# Autodesk Inventor assembly: 1892mm
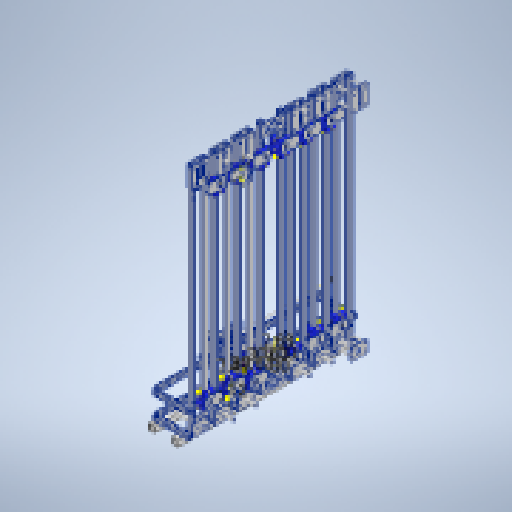
[picture p0: Inventor's stored thumbnail of the model, 512x512]
Saved by Autodesk Inventor 2025 (Build 290162000, 162)
## iProperties
Created: 2025-02-24
Part Number: 1892mm
Document SubType Name: Assembly
Designer: Zhopa
Mass: 1645.37 g
Surface Area: 12511.3 cm^2
Volume: 1061.14 cm^3
Author: Zhopa
## Documents named in this file (24)
- C:\Users\onion\OneDrive - Kyushu University\共有用\工房共有ワンドライブ2024~2025用\ハード\NHK2025\onitsuka\p_a_g\Workspace\Vova\elevator 3\1892mm.iam
- C:\Users\onion\OneDrive - Kyushu University\共有用\工房共有ワンドライブ2024~2025用\ハード\NHK2025\Vova\elevator 3\beams\10x10x600.ipt
- C:\Users\onion\OneDrive - Kyushu University\共有用\工房共有ワンドライブ2024~2025用\ハード\NHK2025\Vova\elevator 3\3D printed\filler_side_fix.ipt
- C:\Users\onion\OneDrive - Kyushu University\共有用\工房共有ワンドライブ2024~2025用\ハード\NHK2025\Vova\elevator 3\cnc\2mm_double_for_pulley.ipt
- C:\Users\onion\OneDrive - Kyushu University\共有用\工房共有ワンドライブ2024~2025用\ハード\NHK2025\Vova\elevator 3\beams\Ф8x40.ipt
- C:\Users\onion\OneDrive - Kyushu University\共有用\工房共有ワンドライブ2024~2025用\ハード\NHK2025\Vova\elevator 3\cnc\2mm_double_for_pulley_v1.ipt
- C:\Users\onion\OneDrive - Kyushu University\共有用\工房共有ワンドライブ2024~2025用\ハード\NHK2025\Vova\elevator 3\cnc\belt_holder_1.ipt
- C:\Users\onion\OneDrive - Kyushu University\共有用\工房共有ワンドライブ2024~2025用\ハード\NHK2025\Vova\elevator 3\cnc\belt_holder_2.ipt
- C:\Users\onion\OneDrive - Kyushu University\共有用\工房共有ワンドライブ2024~2025用\ハード\NHK2025\Vova\elevator 3\cnc\2mm_double_for_pulley_v1_center.ipt
- C:\Users\onion\OneDrive - Kyushu University\共有用\工房共有ワンドライブ2024~2025用\ハード\NHK2025\Vova\elevator 3\bearings\DDLF-1280ZZ.ipt
- C:\Users\onion\OneDrive - Kyushu University\共有用\工房共有ワンドライブ2024~2025用\ハード\NHK2025\Vova\elevator 3\subassemblies\carriage+holder_short.iam
- C:\Users\onion\OneDrive - Kyushu University\共有用\工房共有ワンドライブ2024~2025用\ハード\NHK2025\Vova\elevator 3\beams\10x10x600 - Copy.ipt
- C:\Users\onion\OneDrive - Kyushu University\共有用\工房共有ワンドライブ2024~2025用\ハード\NHK2025\Vova\elevator 3\beams\10x10x60.ipt
- C:\Users\onion\OneDrive - Kyushu University\共有用\工房共有ワンドライブ2024~2025用\ハード\NHK2025\Vova\elevator 3\beams\10x10x431.ipt
- C:\Users\onion\OneDrive - Kyushu University\共有用\工房共有ワンドライブ2024~2025用\ハード\NHK2025\Vova\elevator 3\cnc\motor.ipt
- C:\Users\onion\OneDrive - Kyushu University\共有用\工房共有ワンドライブ2024~2025用\ハード\NHK2025\Vova\elevator 3\motor\M3508.ipt
- C:\Users\onion\OneDrive - Kyushu University\共有用\工房共有ワンドライブ2024~2025用\ハード\NHK2025\Vova\elevator 3\motor\C620.ipt
- C:\Users\onion\OneDrive - Kyushu University\共有用\工房共有ワンドライブ2024~2025用\ハード\NHK2025\Vova\elevator 3\cnc\motor - Copy (2).ipt
- C:\Users\onion\OneDrive - Kyushu University\共有用\工房共有ワンドライブ2024~2025用\ハード\NHK2025\Vova\elevator 3\subassemblies\full short almost works - Copy\Design Accelerator\Spur Gears2.iam
- C:\Users\onion\OneDrive - Kyushu University\共有用\工房共有ワンドライブ2024~2025用\ハード\NHK2025\Vova\elevator 3\beams\Ф8x77.ipt
- C:\Users\onion\OneDrive - Kyushu University\共有用\工房共有ワンドライブ2024~2025用\ハード\NHK2025\Vova\elevator 3\subassemblies\tension.iam
- C:\Users\onion\OneDrive - Kyushu University\共有用\工房共有ワンドライブ2024~2025用\ハード\NHK2025\Vova\elevator 3\cnc\motor - Copy (2) - Copy.ipt
- C:\Users\onion\OneDrive - Kyushu University\共有用\工房共有ワンドライブ2024~2025用\ハード\NHK2025\Vova\elevator 3\3D printed\sapcer34mm.ipt
- C:\Users\onion\OneDrive - Kyushu University\共有用\工房共有ワンドライブ2024~2025用\ハード\NHK2025\Vova\elevator 3\beams\15x15x455.ipt
## Components (101 placed, 23 different names)
1. 10x10x600:9 — 挿入:5, 正接:7, 正接:8, 正接:9, 正接:10, 正接:11, 正接:12, スライダ:1, 挿入:229, 挿入:230, 挿入:231, 挿入:232, 挿入:233, 挿入:234, 挿入:235, 挿入:236
2. filler_side_fix:1 — 挿入:213, 挿入:214
3. filler_side_fix:2 — 挿入:5, 挿入:215, 挿入:216
4. filler_side_fix:3 — 挿入:170, 挿入:171, 挿入:217, 挿入:218
5. filler_side_fix:4 — 挿入:219, 挿入:220
6. 10x10x600:3 — 挿入:24, 挿入:25, 挿入:26, 挿入:27, 挿入:28, 挿入:48, 挿入:49, 挿入:55, 挿入:56, 挿入:58, スライダ:1, 正接:40, 正接:41, 正接:42, 正接:43
7. carriage+holder_short:1 [sub-assembly] — 挿入:24, 挿入:25, 挿入:26, 挿入:27, 正接:7, 正接:8, 正接:9, 正接:10, 正接:11, 正接:12, 挿入:29, 挿入:30, 挿入:31, 挿入:32, 挿入:71, 挿入:72
8. filler_side_fix:5 — 挿入:28, 挿入:29, 挿入:30
9. filler_side_fix:6 — 挿入:31, 挿入:32
10. 2mm_double_for_pulley:1 — 挿入:48, 挿入:168, 挿入:169
11. 2mm_double_for_pulley:2 — 挿入:49, 挿入:51, 挿入:176
12. Ф8x40:1 — 挿入:51
13. 2mm_double_for_pulley_v1:1 — 挿入:55, 挿入:56, 挿入:135, 挿入:172, 挿入:174
14. 2mm_double_for_pulley_v1:2 — 挿入:58, 挿入:60, 挿入:134, 挿入:173, 挿入:175
15. Ф8x40:2 — 挿入:60
16. Ф8x40:3 — 正接:62, 正接:76
17. belt_holder_1:1 — 挿入:71, 挿入:72, 挿入:73, 挿入:74
18. belt_holder_2:1 — 挿入:73, 挿入:74
19. belt_holder_1:2
20. belt_holder_2:2
21. 2mm_double_for_pulley_v1_center:1 — 挿入:182, 挿入:184, 挿入:190, 挿入:192
22. 10x10x600:6 — スライダ:4, 挿入:205, 挿入:206, 挿入:207, 挿入:208, 正接:52, 正接:53, 正接:54, 正接:55
23. 2mm_double_for_pulley:5 — 挿入:198, 挿入:200
24. 2mm_double_for_pulley:6 — 挿入:197, 挿入:199
25. Ф8x40:6
26. 2mm_double_for_pulley_v1:5 — 挿入:138, 挿入:193, 挿入:196
27. 2mm_double_for_pulley_v1:6 — 挿入:140, 挿入:194, 挿入:195
28. Ф8x40:7
29. 10x10x600:8 — スライダ:4, 正接:32, 正接:33, 正接:34, 正接:35, 挿入:225, 挿入:226, 挿入:227, 挿入:228, 挿入:245, 挿入:246, 挿入:247, 挿入:248, 挿入:253, 挿入:254, 挿入:258
30. Ф8x40:9 — 正接:61, 正接:63, 正接:64
31. DDLF-1280ZZ:3 — 挿入:134
32. DDLF-1280ZZ:4 — 挿入:135
33. DDLF-1280ZZ:7 — 挿入:138
34. DDLF-1280ZZ:8 — 挿入:140
35. 2mm_double_for_pulley_v1_center:2 — 挿入:181, 挿入:183, 挿入:189, 挿入:191
36. Ф8x40:13 — 正接:61, 挿入:259
37. 10x10x600 - Copy:1 — 挿入:168, 挿入:169, 挿入:170, 挿入:171, 挿入:172, 挿入:173, 挿入:174, 挿入:175, 挿入:176, 正接:28, 正接:29, 正接:30, 正接:31, 挿入:218, スライダ:5
38. 10x10x600 - Copy:2 — 挿入:181, 挿入:182, 挿入:183, 挿入:184, 挿入:201, 挿入:202, 挿入:203, 挿入:204, 正接:44, 正接:45, 正接:46, 正接:47, スライダ:5
39. 10x10x600 - Copy:3 — 挿入:189, 挿入:190, 挿入:191, 挿入:192, 挿入:209, 挿入:210, 挿入:211, 挿入:212, 正接:48, 正接:49, 正接:50, 正接:51
40. 10x10x600 - Copy:4 — 挿入:193, 挿入:194, 挿入:195, 挿入:196, 挿入:197, 挿入:198, 挿入:199, 挿入:200, 正接:36, 正接:37, 正接:38, 正接:39, 挿入:221, 挿入:222, 挿入:223, 挿入:224
41. carriage+holder_short:2 [sub-assembly] — 挿入:201, 挿入:202, 挿入:203, 挿入:204, 正接:28, 正接:29, 正接:30, 正接:31
42. carriage+holder_short:3 [sub-assembly] — 挿入:205, 挿入:206, 挿入:207, 挿入:208, 正接:32, 正接:33, 正接:34, 正接:35
43. carriage+holder_short:4 [sub-assembly] — 挿入:209, 挿入:210, 挿入:211, 挿入:212, 正接:36, 正接:37, 正接:38, 正接:39
44. carriage+holder_short:5 [sub-assembly] — 挿入:213, 挿入:214, 挿入:215, 挿入:216, 正接:40, 正接:41, 正接:42, 正接:43
45. carriage+holder_short:6 [sub-assembly] — 挿入:217, 挿入:219, 挿入:220, 正接:44, 正接:45, 正接:46, 正接:47
46. carriage+holder_short:7 [sub-assembly] — 挿入:221, 挿入:222, 挿入:223, 挿入:224, 正接:48, 正接:49, 正接:50, 正接:51
47. carriage+holder_short:8 [sub-assembly] — 挿入:225, 挿入:226, 挿入:227, 挿入:228, 正接:52, 正接:53, 正接:54, 正接:55
48. 2mm_double_for_pulley:7 — 挿入:229, 挿入:230, 正接:62, 挿入:237, 挿入:238
49. 2mm_double_for_pulley:8 — 挿入:231, 挿入:232, 挿入:239, 挿入:240
50. 2mm_double_for_pulley_v1:7 — 挿入:233, 挿入:234, 挿入:243, 挿入:244
51. 2mm_double_for_pulley_v1:8 — 挿入:235, 挿入:236, 挿入:241, 挿入:242, 挿入:340
52. 10x10x600:10 — 挿入:237, 挿入:238, 挿入:239, 挿入:240, 挿入:241, 挿入:242, 挿入:243, 挿入:244, 挿入:280, 挿入:281, 挿入:282, 挿入:283, スライダ:6
53. 2mm_double_for_pulley:9 — 挿入:245, 挿入:246, 正接:64, 挿入:249, 挿入:250
54. 2mm_double_for_pulley:10 — 挿入:247, 挿入:248, 正接:63, 挿入:251, 挿入:252
55. 10x10x600:11 — 挿入:249, 挿入:250, 挿入:251, 挿入:252, 挿入:255, 挿入:256, 挿入:257, 挿入:307, 挿入:308, 挿入:309, 挿入:310, スライダ:7
56. 2mm_double_for_pulley_v1:9 — 挿入:253, 挿入:254, 挿入:255, 挿入:256
57. 2mm_double_for_pulley_v1:10 — 挿入:257, 挿入:258, 挿入:259
58. 10x10x600:12 — 挿入:284, 挿入:285, 挿入:286, 挿入:287, スライダ:6, 挿入:336, 挿入:337
59. carriage+holder_short:9 [sub-assembly] — 挿入:280, 挿入:281, 挿入:282, 挿入:283
60. 2mm_double_for_pulley_v1:11
61. 2mm_double_for_pulley_v1:12 — 挿入:334
62. 10x10x600:13 — 挿入:314, 挿入:335, 挿入:338, メイト:3, 角度:1
63. carriage+holder_short:11 [sub-assembly] — 挿入:284, 挿入:285, 挿入:286, 挿入:287
64. 10x10x600:14 — 挿入:292, 挿入:293, 挿入:300, 挿入:301, スライダ:7, 挿入:345, 挿入:346, 挿入:348, 挿入:350
65. Ф8x77:1 — 挿入:306
66. carriage+holder_short:12 [sub-assembly] — 挿入:307, 挿入:308, 挿入:309, 挿入:310
67. carriage+holder_short:13 [sub-assembly]
68. 2mm_double_for_pulley:13 — 挿入:292, 挿入:293, 挿入:296, 挿入:297
69. 2mm_double_for_pulley:14
70. 10x10x600:15 — 挿入:296, 挿入:297, 挿入:302, 挿入:303, 挿入:311, 挿入:312, 挿入:343, 挿入:344, 挿入:347, 挿入:349
71. 2mm_double_for_pulley_v1:13 — 挿入:300, 挿入:301, 挿入:302, 挿入:303
72. 2mm_double_for_pulley_v1:14 — 挿入:306
73. 10x10x60:3 — 挿入:311, 挿入:320, 挿入:352, 挿入:358
74. 10x10x60:4 — 挿入:312, 挿入:353
75. 10x10x60:6 — 挿入:314, 挿入:354, 角度:1
76. motor:1 — 挿入:321, 挿入:322, 挿入:328, 挿入:330, メイト:4, 挿入:355, 挿入:356
77. 10x10x431:2 — 挿入:320, 挿入:342
78. M3508:1 — 挿入:321, 挿入:322, メイト:1
79. C620:1
80. DDLF-1280ZZ:13 — 挿入:328
81. motor - Copy (2):1 — 挿入:330, 挿入:331, 挿入:355
82. DDLF-1280ZZ:14 — 挿入:331
83. Spur Gears:1 [sub-assembly] — メイト:1
84. Ф8x77:2
85. Ф8x77:3 — 挿入:334
86. tension:1 [sub-assembly] — 挿入:335, 挿入:336
87. tension:2 [sub-assembly] — 挿入:337, 挿入:338
88. motor - Copy (2) - Copy:1 — 挿入:356
89. Ф8x40:14 — 挿入:340, 正接:76
90. 10x10x60:7 — 挿入:342, メイト:3, 挿入:351, 挿入:357
91. sapcer34mm:1 — 挿入:343
92. sapcer34mm:2 — 挿入:344
93. sapcer34mm:3 — 挿入:345
94. sapcer34mm:4 — 挿入:346
95. sapcer34mm:5 — 挿入:350
96. sapcer34mm:6 — 挿入:349
97. sapcer34mm:7 — 挿入:348
98. sapcer34mm:8 — 挿入:347
99. 15x15x455:1 — 挿入:351, 挿入:352
100. 10x10x431:3 — 挿入:353, 挿入:354, メイト:4
101. 15x15x455:2 — 挿入:357, 挿入:358
## Relationships (248: Insert 189, Tangent 49, TranslationJoint 5, Mate 4, Angle 1)
- 挿入:5 [Insert]: 10x10x600:9 ↔ filler_side_fix:2
- 挿入:24 [Insert] (8 mm): 10x10x600:3 ↔ carriage+holder_short:1
- 挿入:25 [Insert] (8 mm): 10x10x600:3 ↔ carriage+holder_short:1
- 挿入:26 [Insert] (8 mm): 10x10x600:3 ↔ carriage+holder_short:1
- 挿入:27 [Insert] (8 mm): 10x10x600:3 ↔ carriage+holder_short:1
- 正接:7 [Tangent]: 10x10x600:9 ↔ carriage+holder_short:1
- 正接:8 [Tangent]: 10x10x600:9 ↔ carriage+holder_short:1
- 正接:9 [Tangent]: 10x10x600:9 ↔ carriage+holder_short:1
- 正接:10 [Tangent]: 10x10x600:9 ↔ carriage+holder_short:1
- 正接:11 [Tangent]: 10x10x600:9 ↔ carriage+holder_short:1
- 正接:12 [Tangent]: 10x10x600:9 ↔ carriage+holder_short:1
- 挿入:28 [Insert]: 10x10x600:3 ↔ filler_side_fix:5
- 挿入:29 [Insert]: carriage+holder_short:1 ↔ filler_side_fix:5
- 挿入:30 [Insert]: carriage+holder_short:1 ↔ filler_side_fix:5
- 挿入:31 [Insert]: carriage+holder_short:1 ↔ filler_side_fix:6
- 挿入:32 [Insert]: carriage+holder_short:1 ↔ filler_side_fix:6
- 挿入:48 [Insert]: 10x10x600:3 ↔ 2mm_double_for_pulley:1
- 挿入:49 [Insert]: 10x10x600:3 ↔ 2mm_double_for_pulley:2
- 挿入:51 [Insert] (-2 mm): 2mm_double_for_pulley:2 ↔ Ф8x40:1
- 挿入:55 [Insert]: 10x10x600:3 ↔ 2mm_double_for_pulley_v1:1
- 挿入:56 [Insert]: 10x10x600:3 ↔ 2mm_double_for_pulley_v1:1
- 挿入:58 [Insert]: 10x10x600:3 ↔ 2mm_double_for_pulley_v1:2
- 挿入:60 [Insert]: 2mm_double_for_pulley_v1:2 ↔ Ф8x40:2
- 挿入:71 [Insert]: carriage+holder_short:1 ↔ belt_holder_1:1
- 挿入:72 [Insert]: carriage+holder_short:1 ↔ belt_holder_1:1
- 挿入:73 [Insert] (2 mm): belt_holder_1:1 ↔ belt_holder_2:1
- 挿入:74 [Insert] (2 mm): belt_holder_1:1 ↔ belt_holder_2:1
- [Insert] (2 mm): belt_holder_1:2 ↔ belt_holder_2:2
- [Insert] (2 mm): belt_holder_1:2 ↔ belt_holder_2:2
- [Insert]: 10x10x600:6 ↔ 2mm_double_for_pulley:5
- [Insert]: 10x10x600:6 ↔ 2mm_double_for_pulley:6
- [Insert] (-2 mm): 2mm_double_for_pulley:6 ↔ Ф8x40:6
- [Insert]: 10x10x600:6 ↔ 2mm_double_for_pulley_v1:5
- [Insert]: 10x10x600:6 ↔ 2mm_double_for_pulley_v1:6
- [Insert]: 2mm_double_for_pulley_v1:6 ↔ Ф8x40:7
- 挿入:134 [Insert]: 2mm_double_for_pulley_v1:2 ↔ DDLF-1280ZZ:3
- 挿入:135 [Insert]: 2mm_double_for_pulley_v1:1 ↔ DDLF-1280ZZ:4
- 挿入:138 [Insert]: 2mm_double_for_pulley_v1:5 ↔ DDLF-1280ZZ:7
- 挿入:140 [Insert]: 2mm_double_for_pulley_v1:6 ↔ DDLF-1280ZZ:8
- 挿入:168 [Insert]: 2mm_double_for_pulley:1 ↔ 10x10x600 - Copy:1
- 挿入:169 [Insert]: 2mm_double_for_pulley:1 ↔ 10x10x600 - Copy:1
- 挿入:170 [Insert]: filler_side_fix:3 ↔ 10x10x600 - Copy:1
- 挿入:171 [Insert]: filler_side_fix:3 ↔ 10x10x600 - Copy:1
- 挿入:172 [Insert]: 2mm_double_for_pulley_v1:1 ↔ 10x10x600 - Copy:1
- 挿入:173 [Insert]: 2mm_double_for_pulley_v1:2 ↔ 10x10x600 - Copy:1
- 挿入:174 [Insert]: 2mm_double_for_pulley_v1:1 ↔ 10x10x600 - Copy:1
- 挿入:175 [Insert]: 2mm_double_for_pulley_v1:2 ↔ 10x10x600 - Copy:1
- 挿入:176 [Insert]: 2mm_double_for_pulley:2 ↔ 10x10x600 - Copy:1
- 挿入:181 [Insert]: 2mm_double_for_pulley_v1_center:2 ↔ 10x10x600 - Copy:2
- 挿入:182 [Insert]: 2mm_double_for_pulley_v1_center:1 ↔ 10x10x600 - Copy:2
- 挿入:183 [Insert]: 2mm_double_for_pulley_v1_center:2 ↔ 10x10x600 - Copy:2
- 挿入:184 [Insert]: 2mm_double_for_pulley_v1_center:1 ↔ 10x10x600 - Copy:2
- 挿入:189 [Insert]: 2mm_double_for_pulley_v1_center:2 ↔ 10x10x600 - Copy:3
- 挿入:190 [Insert]: 2mm_double_for_pulley_v1_center:1 ↔ 10x10x600 - Copy:3
- 挿入:191 [Insert]: 2mm_double_for_pulley_v1_center:2 ↔ 10x10x600 - Copy:3
- 挿入:192 [Insert]: 2mm_double_for_pulley_v1_center:1 ↔ 10x10x600 - Copy:3
- 挿入:193 [Insert]: 2mm_double_for_pulley_v1:5 ↔ 10x10x600 - Copy:4
- 挿入:194 [Insert]: 2mm_double_for_pulley_v1:6 ↔ 10x10x600 - Copy:4
- 挿入:195 [Insert]: 2mm_double_for_pulley_v1:6 ↔ 10x10x600 - Copy:4
- 挿入:196 [Insert]: 2mm_double_for_pulley_v1:5 ↔ 10x10x600 - Copy:4
- 挿入:197 [Insert]: 2mm_double_for_pulley:6 ↔ 10x10x600 - Copy:4
- 挿入:198 [Insert]: 2mm_double_for_pulley:5 ↔ 10x10x600 - Copy:4
- 挿入:199 [Insert]: 2mm_double_for_pulley:6 ↔ 10x10x600 - Copy:4
- 挿入:200 [Insert]: 2mm_double_for_pulley:5 ↔ 10x10x600 - Copy:4
- 挿入:201 [Insert] (8 mm): 10x10x600 - Copy:2 ↔ carriage+holder_short:2
- 挿入:202 [Insert] (8 mm): 10x10x600 - Copy:2 ↔ carriage+holder_short:2
- 挿入:203 [Insert] (8 mm): 10x10x600 - Copy:2 ↔ carriage+holder_short:2
- 挿入:204 [Insert] (8 mm): 10x10x600 - Copy:2 ↔ carriage+holder_short:2
- 正接:28 [Tangent]: 10x10x600 - Copy:1 ↔ carriage+holder_short:2
- 正接:29 [Tangent]: 10x10x600 - Copy:1 ↔ carriage+holder_short:2
- 正接:30 [Tangent]: 10x10x600 - Copy:1 ↔ carriage+holder_short:2
- 正接:31 [Tangent]: 10x10x600 - Copy:1 ↔ carriage+holder_short:2
- 挿入:205 [Insert] (8 mm): 10x10x600:6 ↔ carriage+holder_short:3
- 挿入:206 [Insert] (8 mm): 10x10x600:6 ↔ carriage+holder_short:3
- 挿入:207 [Insert] (8 mm): 10x10x600:6 ↔ carriage+holder_short:3
- 挿入:208 [Insert] (8 mm): 10x10x600:6 ↔ carriage+holder_short:3
- 正接:32 [Tangent]: 10x10x600:8 ↔ carriage+holder_short:3
- 正接:33 [Tangent]: 10x10x600:8 ↔ carriage+holder_short:3
- 正接:34 [Tangent]: 10x10x600:8 ↔ carriage+holder_short:3
- 正接:35 [Tangent]: 10x10x600:8 ↔ carriage+holder_short:3
- 挿入:209 [Insert] (8 mm): 10x10x600 - Copy:3 ↔ carriage+holder_short:4
- 挿入:210 [Insert] (8 mm): 10x10x600 - Copy:3 ↔ carriage+holder_short:4
- 挿入:211 [Insert] (8 mm): 10x10x600 - Copy:3 ↔ carriage+holder_short:4
- 挿入:212 [Insert] (8 mm): 10x10x600 - Copy:3 ↔ carriage+holder_short:4
- 正接:36 [Tangent]: 10x10x600 - Copy:4 ↔ carriage+holder_short:4
- 正接:37 [Tangent]: 10x10x600 - Copy:4 ↔ carriage+holder_short:4
- 正接:38 [Tangent]: 10x10x600 - Copy:4 ↔ carriage+holder_short:4
- 正接:39 [Tangent]: 10x10x600 - Copy:4 ↔ carriage+holder_short:4
- 挿入:213 [Insert]: filler_side_fix:1 ↔ carriage+holder_short:5
- 挿入:214 [Insert]: filler_side_fix:1 ↔ carriage+holder_short:5
- 挿入:215 [Insert]: filler_side_fix:2 ↔ carriage+holder_short:5
- 挿入:216 [Insert]: filler_side_fix:2 ↔ carriage+holder_short:5
- 正接:40 [Tangent]: 10x10x600:3 ↔ carriage+holder_short:5
- 正接:41 [Tangent]: 10x10x600:3 ↔ carriage+holder_short:5
- 正接:42 [Tangent]: 10x10x600:3 ↔ carriage+holder_short:5
- 正接:43 [Tangent]: 10x10x600:3 ↔ carriage+holder_short:5
- 挿入:217 [Insert]: filler_side_fix:3 ↔ carriage+holder_short:6
- 挿入:218 [Insert]: filler_side_fix:3 ↔ 10x10x600 - Copy:1
- 挿入:219 [Insert]: filler_side_fix:4 ↔ carriage+holder_short:6
- 挿入:220 [Insert]: filler_side_fix:4 ↔ carriage+holder_short:6
- 正接:44 [Tangent]: 10x10x600 - Copy:2 ↔ carriage+holder_short:6
- 正接:45 [Tangent]: 10x10x600 - Copy:2 ↔ carriage+holder_short:6
- 正接:46 [Tangent]: 10x10x600 - Copy:2 ↔ carriage+holder_short:6
- 正接:47 [Tangent]: 10x10x600 - Copy:2 ↔ carriage+holder_short:6
- 挿入:221 [Insert] (8 mm): 10x10x600 - Copy:4 ↔ carriage+holder_short:7
- 挿入:222 [Insert] (8 mm): 10x10x600 - Copy:4 ↔ carriage+holder_short:7
- 挿入:223 [Insert] (8 mm): 10x10x600 - Copy:4 ↔ carriage+holder_short:7
- 挿入:224 [Insert] (8 mm): 10x10x600 - Copy:4 ↔ carriage+holder_short:7
- 正接:48 [Tangent]: 10x10x600 - Copy:3 ↔ carriage+holder_short:7
- 正接:49 [Tangent]: 10x10x600 - Copy:3 ↔ carriage+holder_short:7
- 正接:50 [Tangent]: 10x10x600 - Copy:3 ↔ carriage+holder_short:7
- 正接:51 [Tangent]: 10x10x600 - Copy:3 ↔ carriage+holder_short:7
- 挿入:225 [Insert] (8 mm): 10x10x600:8 ↔ carriage+holder_short:8
- 挿入:226 [Insert] (8 mm): 10x10x600:8 ↔ carriage+holder_short:8
- 挿入:227 [Insert] (8 mm): 10x10x600:8 ↔ carriage+holder_short:8
- 挿入:228 [Insert] (8 mm): 10x10x600:8 ↔ carriage+holder_short:8
- 正接:52 [Tangent]: 10x10x600:6 ↔ carriage+holder_short:8
- 正接:53 [Tangent]: 10x10x600:6 ↔ carriage+holder_short:8
- 正接:54 [Tangent]: 10x10x600:6 ↔ carriage+holder_short:8
- 正接:55 [Tangent]: 10x10x600:6 ↔ carriage+holder_short:8
- スライダ:1 [TranslationJoint] (16 mm): 10x10x600:9 ↔ 10x10x600:3
- スライダ:4 [TranslationJoint] (16 mm): 10x10x600:6 ↔ 10x10x600:8
- スライダ:5 [TranslationJoint] (16 mm): 10x10x600 - Copy:1 ↔ 10x10x600 - Copy:2
- 正接:61 [Tangent] (560.96 mm): Ф8x40:9 ↔ Ф8x40:13
- 挿入:229 [Insert]: 10x10x600:9 ↔ 2mm_double_for_pulley:7
- 挿入:230 [Insert]: 10x10x600:9 ↔ 2mm_double_for_pulley:7
- 挿入:231 [Insert]: 10x10x600:9 ↔ 2mm_double_for_pulley:8
- 挿入:232 [Insert]: 10x10x600:9 ↔ 2mm_double_for_pulley:8
- 正接:62 [Tangent]: Ф8x40:3 ↔ 2mm_double_for_pulley:7
- 挿入:233 [Insert]: 10x10x600:9 ↔ 2mm_double_for_pulley_v1:7
- 挿入:234 [Insert]: 10x10x600:9 ↔ 2mm_double_for_pulley_v1:7
- 挿入:235 [Insert]: 10x10x600:9 ↔ 2mm_double_for_pulley_v1:8
- 挿入:236 [Insert]: 10x10x600:9 ↔ 2mm_double_for_pulley_v1:8
- 挿入:237 [Insert]: 2mm_double_for_pulley:7 ↔ 10x10x600:10
- 挿入:238 [Insert]: 2mm_double_for_pulley:7 ↔ 10x10x600:10
- 挿入:239 [Insert]: 2mm_double_for_pulley:8 ↔ 10x10x600:10
- 挿入:240 [Insert]: 2mm_double_for_pulley:8 ↔ 10x10x600:10
- 挿入:241 [Insert]: 2mm_double_for_pulley_v1:8 ↔ 10x10x600:10
- 挿入:242 [Insert]: 2mm_double_for_pulley_v1:8 ↔ 10x10x600:10
- 挿入:243 [Insert]: 2mm_double_for_pulley_v1:7 ↔ 10x10x600:10
- 挿入:244 [Insert]: 2mm_double_for_pulley_v1:7 ↔ 10x10x600:10
- 挿入:245 [Insert]: 10x10x600:8 ↔ 2mm_double_for_pulley:9
- 挿入:246 [Insert]: 10x10x600:8 ↔ 2mm_double_for_pulley:9
- 挿入:247 [Insert]: 10x10x600:8 ↔ 2mm_double_for_pulley:10
- 挿入:248 [Insert]: 10x10x600:8 ↔ 2mm_double_for_pulley:10
- 正接:63 [Tangent]: Ф8x40:9 ↔ 2mm_double_for_pulley:10
- 正接:64 [Tangent]: Ф8x40:9 ↔ 2mm_double_for_pulley:9
- 挿入:249 [Insert]: 2mm_double_for_pulley:9 ↔ 10x10x600:11
- 挿入:250 [Insert]: 2mm_double_for_pulley:9 ↔ 10x10x600:11
- 挿入:251 [Insert]: 2mm_double_for_pulley:10 ↔ 10x10x600:11
- 挿入:252 [Insert]: 2mm_double_for_pulley:10 ↔ 10x10x600:11
- 挿入:253 [Insert]: 10x10x600:8 ↔ 2mm_double_for_pulley_v1:9
- 挿入:254 [Insert]: 10x10x600:8 ↔ 2mm_double_for_pulley_v1:9
- 挿入:255 [Insert]: 10x10x600:11 ↔ 2mm_double_for_pulley_v1:9
- 挿入:256 [Insert]: 10x10x600:11 ↔ 2mm_double_for_pulley_v1:9
- 挿入:257 [Insert]: 10x10x600:11 ↔ 2mm_double_for_pulley_v1:10
- 挿入:258 [Insert]: 10x10x600:8 ↔ 2mm_double_for_pulley_v1:10
- 挿入:259 [Insert]: Ф8x40:13 ↔ 2mm_double_for_pulley_v1:10
- [Tangent]: 10x10x600:12 ↔ carriage+holder_short:9
- [Tangent]: 10x10x600:12 ↔ carriage+holder_short:9
- [Tangent]: 10x10x600:12 ↔ carriage+holder_short:9
- [Tangent]: 10x10x600:12 ↔ carriage+holder_short:9
- [Tangent]: 10x10x600:12 ↔ carriage+holder_short:9
- [Tangent]: 10x10x600:12 ↔ carriage+holder_short:9
- [Insert]: 10x10x600:12 ↔ 2mm_double_for_pulley_v1:11
- [Insert]: 10x10x600:12 ↔ 2mm_double_for_pulley_v1:11
- [Insert]: 10x10x600:12 ↔ 2mm_double_for_pulley_v1:12
- [Insert]: 10x10x600:12 ↔ 2mm_double_for_pulley_v1:12
- [Insert]: 2mm_double_for_pulley_v1:12 ↔ 10x10x600:13
- [Insert]: 2mm_double_for_pulley_v1:12 ↔ 10x10x600:13
- [Insert]: 2mm_double_for_pulley_v1:11 ↔ 10x10x600:13
- [Insert]: 2mm_double_for_pulley_v1:11 ↔ 10x10x600:13
- 挿入:280 [Insert] (8 mm): 10x10x600:10 ↔ carriage+holder_short:9
- 挿入:281 [Insert] (8 mm): 10x10x600:10 ↔ carriage+holder_short:9
- 挿入:282 [Insert] (8 mm): 10x10x600:10 ↔ carriage+holder_short:9
- 挿入:283 [Insert] (8 mm): 10x10x600:10 ↔ carriage+holder_short:9
- 挿入:284 [Insert] (8 mm): 10x10x600:12 ↔ carriage+holder_short:11
- 挿入:285 [Insert] (8 mm): 10x10x600:12 ↔ carriage+holder_short:11
- 挿入:286 [Insert] (8 mm): 10x10x600:12 ↔ carriage+holder_short:11
- 挿入:287 [Insert] (8 mm): 10x10x600:12 ↔ carriage+holder_short:11
- [Tangent]: 10x10x600:14 ↔ carriage+holder_short:12
- [Tangent]: 10x10x600:14 ↔ carriage+holder_short:12
- [Tangent]: 10x10x600:14 ↔ carriage+holder_short:12
- [Tangent]: 10x10x600:14 ↔ carriage+holder_short:12
- [Insert] (8 mm): 10x10x600:14 ↔ carriage+holder_short:13
- [Insert] (8 mm): 10x10x600:14 ↔ carriage+holder_short:13
- [Insert] (8 mm): 10x10x600:14 ↔ carriage+holder_short:13
- [Insert] (8 mm): 10x10x600:14 ↔ carriage+holder_short:13
- 挿入:292 [Insert] (34 mm): 10x10x600:14 ↔ 2mm_double_for_pulley:13
- 挿入:293 [Insert] (34 mm): 10x10x600:14 ↔ 2mm_double_for_pulley:13
- [Insert]: 10x10x600:14 ↔ 2mm_double_for_pulley:14
- [Insert]: 10x10x600:14 ↔ 2mm_double_for_pulley:14
- 挿入:296 [Insert] (34 mm): 2mm_double_for_pulley:13 ↔ 10x10x600:15
- 挿入:297 [Insert] (34 mm): 2mm_double_for_pulley:13 ↔ 10x10x600:15
- [Insert]: 2mm_double_for_pulley:14 ↔ 10x10x600:15
- [Insert]: 2mm_double_for_pulley:14 ↔ 10x10x600:15
- 挿入:300 [Insert] (34 mm): 10x10x600:14 ↔ 2mm_double_for_pulley_v1:13
- 挿入:301 [Insert] (34 mm): 10x10x600:14 ↔ 2mm_double_for_pulley_v1:13
- 挿入:302 [Insert] (34 mm): 10x10x600:15 ↔ 2mm_double_for_pulley_v1:13
- 挿入:303 [Insert] (34 mm): 10x10x600:15 ↔ 2mm_double_for_pulley_v1:13
- [Insert]: 10x10x600:15 ↔ 2mm_double_for_pulley_v1:14
- [Insert]: 10x10x600:14 ↔ 2mm_double_for_pulley_v1:14
- 挿入:306 [Insert] (-50 mm): Ф8x77:1 ↔ 2mm_double_for_pulley_v1:14
- 挿入:307 [Insert] (8 mm): 10x10x600:11 ↔ carriage+holder_short:12
- 挿入:308 [Insert] (8 mm): 10x10x600:11 ↔ carriage+holder_short:12
- 挿入:309 [Insert] (8 mm): 10x10x600:11 ↔ carriage+holder_short:12
- 挿入:310 [Insert] (8 mm): 10x10x600:11 ↔ carriage+holder_short:12
- スライダ:6 [TranslationJoint] (16 mm): 10x10x600:10 ↔ 10x10x600:12
- スライダ:7 [TranslationJoint] (16 mm): 10x10x600:11 ↔ 10x10x600:14
- 挿入:311 [Insert]: 10x10x600:15 ↔ 10x10x60:3
- 挿入:312 [Insert]: 10x10x600:15 ↔ 10x10x60:4
- 挿入:314 [Insert]: 10x10x600:13 ↔ 10x10x60:6
- 挿入:320 [Insert]: 10x10x60:3 ↔ 10x10x431:2
- 挿入:321 [Insert]: motor:1 ↔ M3508:1
- 挿入:322 [Insert]: motor:1 ↔ M3508:1
- 挿入:328 [Insert]: motor:1 ↔ DDLF-1280ZZ:13
- 挿入:330 [Insert] (34 mm): motor:1 ↔ motor - Copy (2):1
- 挿入:331 [Insert]: motor - Copy (2):1 ↔ DDLF-1280ZZ:14
- [Insert] (14 mm): DDLF-1280ZZ:14 ↔ Ф8x77:2
- メイト:1 [Mate]: M3508:1 ↔ Spur Gears:1
- [Mate]: Spur Gears:1 ↔ Ф8x77:2
- 挿入:334 [Insert] (-20 mm): 2mm_double_for_pulley_v1:12 ↔ Ф8x77:3
- 挿入:335 [Insert]: 10x10x600:13 ↔ tension:1
- 挿入:336 [Insert]: 10x10x600:12 ↔ tension:1
- 挿入:337 [Insert]: 10x10x600:12 ↔ tension:2
- 挿入:338 [Insert]: 10x10x600:13 ↔ tension:2
- 挿入:340 [Insert]: 2mm_double_for_pulley_v1:8 ↔ Ф8x40:14
- 正接:76 [Tangent] (551.18 mm): Ф8x40:3 ↔ Ф8x40:14
- 挿入:342 [Insert]: 10x10x431:2 ↔ 10x10x60:7
- メイト:3 [Mate]: 10x10x600:13 ↔ 10x10x60:7
- 挿入:343 [Insert]: 10x10x600:15 ↔ sapcer34mm:1
- 挿入:344 [Insert]: 10x10x600:15 ↔ sapcer34mm:2
- 挿入:345 [Insert]: 10x10x600:14 ↔ sapcer34mm:3
- 挿入:346 [Insert]: 10x10x600:14 ↔ sapcer34mm:4
- 挿入:347 [Insert]: 10x10x600:15 ↔ sapcer34mm:8
- 挿入:348 [Insert]: 10x10x600:14 ↔ sapcer34mm:7
- 挿入:349 [Insert]: 10x10x600:15 ↔ sapcer34mm:6
- 挿入:350 [Insert]: 10x10x600:14 ↔ sapcer34mm:5
- 挿入:351 [Insert]: 10x10x60:7 ↔ 15x15x455:1
- 挿入:352 [Insert]: 10x10x60:3 ↔ 15x15x455:1
- 挿入:353 [Insert]: 10x10x60:4 ↔ 10x10x431:3
- 挿入:354 [Insert]: 10x10x60:6 ↔ 10x10x431:3
- メイト:4 [Mate]: motor:1 ↔ 10x10x431:3
- 挿入:355 [Insert] (34 mm): motor:1 ↔ motor - Copy (2):1
- 角度:1 [Angle] (-90 deg): 10x10x600:13 ↔ 10x10x60:6
- 挿入:356 [Insert] (45 mm): motor:1 ↔ motor - Copy (2) - Copy:1
- 挿入:357 [Insert]: 10x10x60:7 ↔ 15x15x455:2
- 挿入:358 [Insert]: 10x10x60:3 ↔ 15x15x455:2
## Named parameters: d94_d92 = 2 mm, d95_d93 = 2 mm, d131_d76 = 0 mm, d133_d78 = 0 mm, d134_d79 = 0 mm, d135_d66 = 0 mm, d138_d69 = 0 mm, d139_d70 = -2 mm, d404_d37 = 0 mm, d405_d38 = 0 mm, d406_d39 = 0 mm, d407_d40 = 0 mm, d408_d41 = 0 mm, d409_d42 = 0 mm, d415_d371 = 0 mm, d416_d372 = 0 mm, d417_d373 = 0 mm, d418_d374 = 0 mm, d419_d379 = 0 mm, d420_d380 = 0 mm, d421_d381 = 0 mm, d422_d382 = 0 mm, d436_d318 = 8 mm, d437_d319 = 8 mm, d438_d320 = 8 mm, d439_d321 = 8 mm, d440_d282 = 0 mm, d441_d283 = 0 mm, d442_d284 = 0 mm, d443_d285 = 0 mm, d444_d394 = 34 mm, d445_d395 = 34 mm, d446_d396 = 34 mm, d447_d397 = 0 mm, d448_d398 = 0 mm, d449_d399 = -50 mm, d450_d390 = 34 mm, d451_d391 = 0 mm, d452_d392 = 0 mm, d453_d393 = 34 mm, d456_d389 = 34 mm, d457_d383 = 34 mm, d458_d384 = 34 mm, d459_d385 = 0 mm, d460_d386 = 0 mm
